# Autodesk Inventor assembly: Diff_Assembly_V1
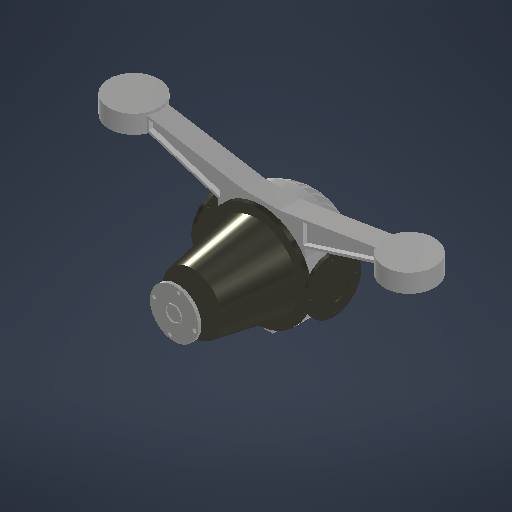
[picture p0: Inventor's stored thumbnail of the model, 512x512]
Saved by Autodesk Inventor 2026.1 (Build 301233000, 233)
## iProperties
Created: 2026-08-05
Part Number: Diff_Assembly_V1
Document SubType Name: Assembly
Designer: share
Author: share
## Documents named in this file (4)
- C:\Users\share\OneDrive\Documents\Personal Projects\GOGO Kart\CAD\GOGO_KART_FSAE\Drivetrain\Diff_Assembly_V1.iam
- C:\Users\share\OneDrive\Documents\Personal Projects\GOGO Kart\CAD\GOGO_KART_FSAE\Drivetrain\Diff V2.ipt
- C:\Users\share\OneDrive\Documents\Personal Projects\GOGO Kart\CAD\GOGO_KART_FSAE\Drivetrain\Diff_CV_Output_V1.ipt
- C:\Users\share\OneDrive\Documents\Personal Projects\GOGO Kart\CAD\GOGO_KART_FSAE\Drivetrain\Diff_Driveshaft_Output_V1.ipt
## Components (4 placed, 3 different names)
1. Diff V2:1 — Mate:1, Flush:1, Flush:2, Flush:3, Mate:2, Mate:4, Flush:5
2. Diff_CV_Output_V1:1 — Mate:1, Flush:4
3. Diff_CV_Output_V1:2 — Mate:2, Mate:3
4. Diff_Driveshaft_Output_V1:1 — Mate:4, Flush:5
## Relationships (9: Flush 5, Mate 4)
- Mate:1: Diff V2:1 ↔ Diff_CV_Output_V1:1
- Flush:1: Diff V2:1
- Flush:2: Diff V2:1
- Flush:3: Diff V2:1
- Mate:2: Diff V2:1 ↔ Diff_CV_Output_V1:2
- Mate:3 (-125 mm): Diff_CV_Output_V1:2
- Flush:4 (125 mm): Diff_CV_Output_V1:1
- Mate:4: Diff V2:1 ↔ Diff_Driveshaft_Output_V1:1
- Flush:5 (160 mm): Diff V2:1 ↔ Diff_Driveshaft_Output_V1:1
